# Autodesk Inventor assembly: assembled
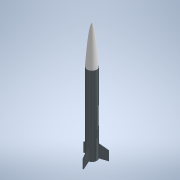
[picture p0: Inventor's stored thumbnail of the model, 180x180]
Saved by Autodesk Inventor 2020.3 (Build 243373000, 373)
## iProperties
Created: 2021-03-15
Part Number: assembled
Document SubType Name: Assembly
Designer: 0x6f736f646f
Author: 0x6f736f646f
## Documents named in this file (7)
- C:\Users\0x6f736f646f\OneDrive\Documents\Inventor\Nakuja project\assembled.iam
- C:\Users\0x6f736f646f\OneDrive\Documents\Inventor\Nakuja project\noseAssembly.iam
- C:\Users\0x6f736f646f\OneDrive\Documents\Inventor\Nakuja project\electronicsbay.ipt
- C:\Users\0x6f736f646f\OneDrive\Documents\Inventor\Nakuja project\extraTube.ipt
- C:\Users\0x6f736f646f\OneDrive\Documents\Inventor\Nakuja project\launchlug.ipt
- C:\Users\0x6f736f646f\OneDrive\Documents\Inventor\Nakuja project\payloadchamber.ipt
- C:\Users\0x6f736f646f\OneDrive\Documents\Inventor\Nakuja project\tail.ipt
## Components (6 placed, 6 different names)
1. electronicsbay:1 — Mate:1, Rigid:1
2. extraTube:1 — Mate:2, Mate:3, Mate:4, Mate:5
3. launchlug:1 — Mate:8, Mate:9
4. payloadchamber:1 — Mate:1, Mate:2, Rigid:1, Mate:5, Cylindrical:1
5. tail:1 — Mate:3, Mate:4, Mate:8, Mate:9
6. noseAssembly:1 [sub-assembly] — Cylindrical:1
## Relationships (9: Mate 7, WeldJoint 1, CylindricalJoint 1)
- Mate:1: electronicsbay:1 ↔ payloadchamber:1
- Mate:2: extraTube:1 ↔ payloadchamber:1
- Rigid:1 [WeldJoint]: electronicsbay:1 ↔ payloadchamber:1
- Mate:3: extraTube:1 ↔ tail:1
- Mate:4: extraTube:1 ↔ tail:1
- Mate:5: extraTube:1 ↔ payloadchamber:1
- Mate:8 (33.6 mm): launchlug:1 ↔ tail:1
- Mate:9: launchlug:1 ↔ tail:1
- Cylindrical:1: payloadchamber:1 ↔ noseAssembly:1
